# Autodesk Inventor assembly: NEMA 17 T8x8 Assembly
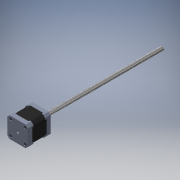
[picture p0: Inventor's stored thumbnail of the model, 180x180]
Saved by Autodesk Inventor 2016 (Build 200138000, 138)
## iProperties
Created: 2017-02-12
Part Number: NEMA 17 T8x8 Assembly
Document SubType Name: Assembly
Designer: Scott
Author: Scott
## Documents named in this file (3)
- E:\Scott Projects\3D Printing\CoreXY\NEMA 17 T8x8 Assembly.iam
- E:\Scott Projects\3D Printing\CoreXY\NEMA 17 Stepper Motor Assembly.iam
- E:\Scott Projects\3D Printing\CoreXY\T8x8 Lead Screw.ipt
## Components (2 placed, 2 different names)
1. NEMA 17 Stepper Motor Assembly:1 [sub-assembly] — Insert:1
2. T8x8 Lead Screw:1 — Insert:1
## Relationships (1: Insert 1)
- Insert:1: NEMA 17 Stepper Motor Assembly:1 ↔ T8x8 Lead Screw:1
